# Autodesk Inventor assembly: Krzyżyk
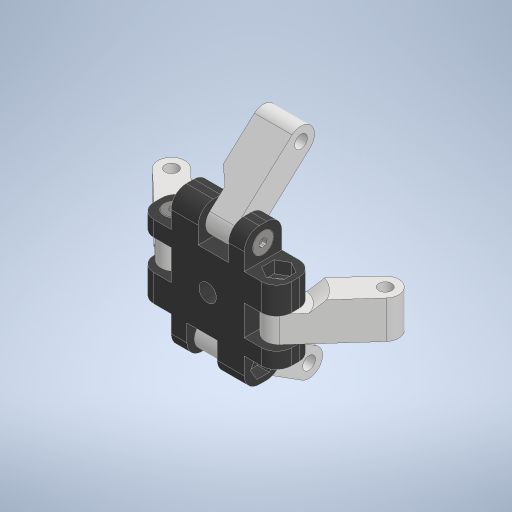
[picture p0: Inventor's stored thumbnail of the model, 512x512]
Saved by Autodesk Inventor 2023 (Build 270158000, 158)
## iProperties
Created: 2023-06-03
Part Number: Krzyżyk
Document SubType Name: Assembly
Designer: Kamil
Author: Kamil
## Documents named in this file (4)
- C:\Users\Kamil\Desktop\KONARM_2\chwytak\Krzyżyk.iam
- C:\Users\Kamil\Desktop\KONARM_2\chwytak\ArmMuscle.ipt
- C:\Users\Kamil\Desktop\KONARM_2\chwytak\GripperMotorHinges.ipt
- C:\Users\Kamil\Documents\Inventor\Content Center Files\R2023\pl-PL\ASME ANSI B18.3.5M(2)\ASME_ANSI B18.3.5M - M3x20(2).ipt
## Components (7 placed, 3 different names)
1. GripperMotorHinges:1 — Zestawiające:1, Zestawiające:2, Zestawiające:3, Zestawiające:4, Zestawiające:5, Zestawiające:6, Zestawiające:7, Zestawiające:8, Zestawiające:9, Zestawiające:10
2. ArmMuscle:1 — Zestawiające:1, Zestawiające:2
3. ArmMuscle:2 — Zestawiające:3, Zestawiające:4
4. ArmMuscle:3 — Zestawiające:5, Zestawiające:6
5. ArmMuscle:4 — Zestawiające:7, Zestawiające:8
6. Wkręt z łbem stożkowym, wpuszczanym, z gniazdem sześciokątnym ciągnionym - metryczny M3x20:1 — Zestawiające:10
7. Wkręt z łbem stożkowym, wpuszczanym, z gniazdem sześciokątnym ciągnionym - metryczny M3x20:2 — Zestawiające:9
## Relationships (10: Mate 10)
- Zestawiające:1 [Mate] (0.5 mm): GripperMotorHinges:1 ↔ ArmMuscle:1
- Zestawiające:2 [Mate]: GripperMotorHinges:1 ↔ ArmMuscle:1
- Zestawiające:3 [Mate] (0.5 mm): GripperMotorHinges:1 ↔ ArmMuscle:2
- Zestawiające:4 [Mate]: GripperMotorHinges:1 ↔ ArmMuscle:2
- Zestawiające:5 [Mate] (0.5 mm): GripperMotorHinges:1 ↔ ArmMuscle:3
- Zestawiające:6 [Mate]: GripperMotorHinges:1 ↔ ArmMuscle:3
- Zestawiające:7 [Mate] (0.5 mm): GripperMotorHinges:1 ↔ ArmMuscle:4
- Zestawiające:8 [Mate]: GripperMotorHinges:1 ↔ ArmMuscle:4
- Zestawiające:9 [Mate]: GripperMotorHinges:1 ↔ Wkręt z łbem stożkowym, wpuszczanym, z gniazdem sześciokątnym ciągnionym - metryczny M3x20:2
- Zestawiające:10 [Mate]: GripperMotorHinges:1 ↔ Wkręt z łbem stożkowym, wpuszczanym, z gniazdem sześciokątnym ciągnionym - metryczny M3x20:1
